# Autodesk Inventor assembly: Cat_head
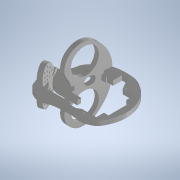
[picture p0: Inventor's stored thumbnail of the model, 180x180]
Saved by Autodesk Inventor 2022 (Build 260153000, 153)
## iProperties
Created: 2023-02-10
Part Number: Cat_head
Document SubType Name: Assembly
Designer: scott
Author: scott
## Documents named in this file (4)
- C:\Users\scott\OneDrive\Documents\Cat project\Git_repository\Flinders_OpenCat\CAD components\Cat_head.iam
- C:\Users\scott\OneDrive\Documents\Cat project\Git_repository\Flinders_OpenCat\CAD components\NybbleDIY\Imported Components\Skull\Skull.ipt
- C:\Users\scott\OneDrive\Documents\Cat project\Git_repository\Flinders_OpenCat\CAD components\NybbleDIY\Imported Components\Whiskers\Whiskers.ipt
- C:\Users\scott\OneDrive\Documents\Cat project\Git_repository\Flinders_OpenCat\CAD components\NybbleDIY\Imported Components\Eyes\Eyes.ipt
## Components (3 placed, 3 different names)
1. Skull:1 — Mate:1, Mate:2, Mate:3, Mate:4, Mate:5
2. Whiskers:1 — Mate:1, Mate:2, Mate:3
3. Eyes:1 — Mate:4, Mate:5
## Relationships (5: Mate 5)
- Mate:1: Skull:1 ↔ Whiskers:1
- Mate:2: Skull:1 ↔ Whiskers:1
- Mate:3: Skull:1 ↔ Whiskers:1
- Mate:4: Skull:1 ↔ Eyes:1
- Mate:5: Skull:1 ↔ Eyes:1
